# Autodesk Inventor assembly: BBP
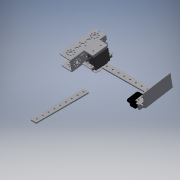
[picture p0: Inventor's stored thumbnail of the model, 180x180]
Saved by Autodesk Inventor 2016 (Build 200138000, 138)
## iProperties
Created: 2016-09-30
Part Number: BBP
Document SubType Name: Assembly
Designer: Delta
Author: Delta
## Documents named in this file (11)
- C:\Robotics\CAD\2016-17_CAD\BBP.iam
- C:\Robotics\CAD\COTSParts\Tetrix\Tetrix channel 160mm.ipt
- C:\Robotics\CAD\COTSParts\Tetrix\Tetrix bracket - single servo.ipt
- C:\Robotics\CAD\COTSParts\Actobotics\585 parts\585382.ipt
- C:\Robotics\CAD\COTSParts\Tetrix\Tetrix servo 180.ipt
- C:\Robotics\CAD\2015-16_CAD\Part5.ipt
- C:\Robotics\CAD\2015-16_CAD\Part6.ipt
- C:\Robotics\CAD\2015-16_CAD\Tetrix angle 144mm_3in.ipt
- C:\Robotics\CAD\COTSParts\ModernRobotics\45-2006_ODS.ipt
- C:\Robotics\CAD\COTSParts\Tetrix\Tetrix flat bar 7 in.ipt
- C:\Robotics\CAD\COTSParts\Tetrix\Tetrix flat bar 5.75.ipt
## Components (11 placed, 10 different names)
1. Tetrix channel 160mm:2 — Insert:16
2. Tetrix bracket - single servo:1 — Mate:1, Flush:1, Flush:2, Insert:16
3. Tetrix servo 180:1 — Mate:1, Flush:1, Flush:2
4. 585382:5 — Mate:4, Insert:15, Insert:17, Insert:18
5. Part5:1 — Insert:19
6. Part6:1 — Mate:2, Flush:5, Flush:6
7. Tetrix angle 144mm_3in:1 — Flush:7, Flush:8, Mate:3, Insert:17, Flush:9
8. Tetrix angle 144mm_3in:2 — Mate:2, Flush:5, Flush:6, Flush:7, Flush:8, Mate:3, Flush:9
9. 45-2006_ODS:1 — Mate:4, Insert:15
10. Tetrix flat bar 7 in:1 — Insert:18, Insert:19
11. Tetrix flat bar 5.75:1
## Relationships (16: Flush 7, Insert 5, Mate 4)
- Mate:1 (5.3594 mm): Tetrix bracket - single servo:1 ↔ Tetrix servo 180:1
- Flush:1: Tetrix bracket - single servo:1 ↔ Tetrix servo 180:1
- Flush:2: Tetrix bracket - single servo:1 ↔ Tetrix servo 180:1
- Mate:2: Part6:1 ↔ Tetrix angle 144mm_3in:2
- Flush:5: Part6:1 ↔ Tetrix angle 144mm_3in:2
- Flush:6: Part6:1 ↔ Tetrix angle 144mm_3in:2
- Flush:7: Tetrix angle 144mm_3in:1 ↔ Tetrix angle 144mm_3in:2
- Flush:8: Tetrix angle 144mm_3in:1 ↔ Tetrix angle 144mm_3in:2
- Mate:3: Tetrix angle 144mm_3in:1 ↔ Tetrix angle 144mm_3in:2
- Mate:4: 585382:5 ↔ 45-2006_ODS:1
- Insert:15: 585382:5 ↔ 45-2006_ODS:1
- Insert:16: Tetrix channel 160mm:2 ↔ Tetrix bracket - single servo:1
- Insert:17: 585382:5 ↔ Tetrix angle 144mm_3in:1
- Flush:9 (4.3434 mm): Tetrix angle 144mm_3in:1 ↔ Tetrix angle 144mm_3in:2
- Insert:18: 585382:5 ↔ Tetrix flat bar 7 in:1
- Insert:19: Part5:1 ↔ Tetrix flat bar 7 in:1
